# Autodesk Inventor assembly: zlozenie
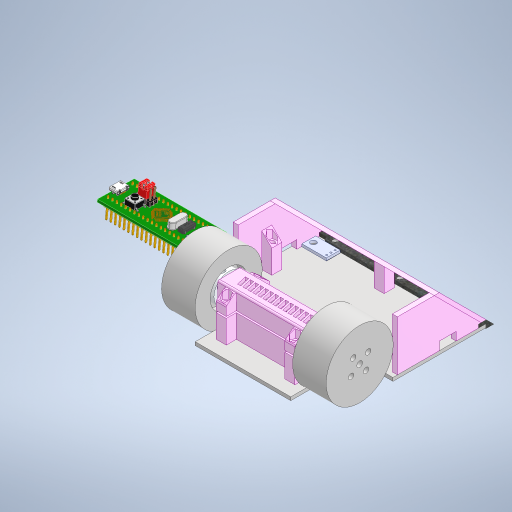
[picture p0: Inventor's stored thumbnail of the model, 512x512]
Saved by Autodesk Inventor 2023 (Build 270158000, 158)
## iProperties
Created: 2023-03-01
Part Number: zlozenie
Document SubType Name: Assembly
Designer: Eryk
Author: Eryk
## Documents named in this file (11)
- C:\Users\Eryk\Documents\PEM\assembly.iam
- C:\Users\Eryk\Documents\PEM\motor_mount.ipt
- C:\Users\Eryk\Documents\PEM\base.ipt
- C:\Users\Eryk\Documents\PEM\Pololu-Micro-Metal-Gearmotor.ipt
- C:\Users\Eryk\Documents\PEM\front_assembly.iam
- C:\Users\Eryk\Documents\PEM\Plog2.ipt
- C:\Users\Eryk\Documents\PEM\wheel.ipt
- C:\Users\Eryk\Documents\PEM\motor_hub.ipt
- C:\Users\Eryk\Documents\PEM\Blue Pill STM32.iam
- C:\Users\Eryk\Documents\PEM\QRE1113 DIGITAL.ipt
- C:\Users\Eryk\Documents\PEM\Proximity Sensor.ipt
## Components (13 placed, 10 different names)
1. base:1 — Mate:12, Mate:13, Flush:1, Mate:14, Mate:15, Mate:20
2. motor_mount:1 — Mate:12, Mate:16, Mate:17, Mate:18, Mate:19
3. Pololu-Micro-Metal-Gearmotor:1 — Mate:16, Mate:17, Insert:1
4. Pololu-Micro-Metal-Gearmotor:2 — Mate:18, Mate:19, Insert:2
5. front_assembly:1 [sub-assembly] — Mate:14, Mate:15
6. Plog2:1 — Mate:13, Flush:1
7. wheel:1 — Rotational:2
8. motor_hub:1 — Insert:2, Rotational:2
9. wheel:2 — Rotational:1
10. motor_hub:2 — Insert:1, Rotational:1
11. Blue Pill STM32:1 [sub-assembly]
12. QRE1113 DIGITAL:1 — Mate:20
13. Proximity Sensor:1
## Relationships (14: Mate 9, Insert 2, RevoluteJoint 2, Flush 1)
- Mate:12: base:1 ↔ motor_mount:1
- Mate:13: base:1 ↔ Plog2:1
- Flush:1: base:1 ↔ Plog2:1
- Mate:14: base:1 ↔ front_assembly:1
- Mate:15: base:1 ↔ front_assembly:1
- Mate:16: motor_mount:1 ↔ Pololu-Micro-Metal-Gearmotor:1
- Mate:17: motor_mount:1 ↔ Pololu-Micro-Metal-Gearmotor:1
- Mate:18: motor_mount:1 ↔ Pololu-Micro-Metal-Gearmotor:2
- Mate:19: motor_mount:1 ↔ Pololu-Micro-Metal-Gearmotor:2
- Insert:1: Pololu-Micro-Metal-Gearmotor:1 ↔ motor_hub:2
- Rotational:1 [RevoluteJoint]: wheel:2 ↔ motor_hub:2
- Insert:2: Pololu-Micro-Metal-Gearmotor:2 ↔ motor_hub:1
- Rotational:2 [RevoluteJoint]: wheel:1 ↔ motor_hub:1
- Mate:20: base:1 ↔ QRE1113 DIGITAL:1
